# Autodesk Inventor assembly: 60T x 18mm Wide VersaPulley Kit (HTD 5mm, VersaKeys) (217-3200)
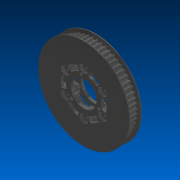
[picture p0: Inventor's stored thumbnail of the model, 180x180]
Saved by Autodesk Inventor 2022.2 (Build 262287000, 287)
## iProperties
Created: 2013-12-06
Part Number: 60T x 18mm Wide VersaPulley Kit (HTD 5mm, VersaKeys) (217-3200)
Description: STEP AP214
Document SubType Name: Assembly
Designer: omard
Sending System: SolidWorks 2013
Preprocessor: SwSTEP 2.0
Title: 217-3200-STEP.STEP
Revision Number: ANY
## Documents named in this file (2)
- D:\omard\OneDrive - Auburn University\BasketBall Shooting Robot\VEX Parts\60T x 18mm Wide VersaPulley Kit (HTD 5mm, VersaKeys) (217-3200).iam
- D:\omard\OneDrive - Auburn University\BasketBall Shooting Robot\VEX Parts\Components\217-3200-001 Rev3.ipt
## Components (2 placed, 2 different names)
1. 217-3200-001 Rev3_1 — Mate:1, Mate:2, Mate:3
2. 217-3200-001 Rev3_2 — Mate:1, Mate:2, Mate:3
## Relationships (3: Mate 3)
- Mate:1: 217-3200-001 Rev3_1 ↔ 217-3200-001 Rev3_2
- Mate:2: 217-3200-001 Rev3_1 ↔ 217-3200-001 Rev3_2
- Mate:3: 217-3200-001 Rev3_1 ↔ 217-3200-001 Rev3_2
